# Autodesk Inventor assembly: BobbinGuide
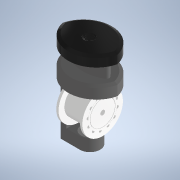
[picture p0: Inventor's stored thumbnail of the model, 180x180]
Saved by Autodesk Inventor 2022 (Build 260153000, 153)
## iProperties
Created: 2020-03-09
Part Number: BobbinGuide
Document SubType Name: Assembly
Designer: elmar
Author: elmar
## Documents named in this file (6)
- C:\repo\FourWireBraidingMachine\MetalCableBraider\Carriage.iam
- C:\repo\FourWireBraidingMachine\MetalCableBraider\CarriagePlate.ipt
- C:\repo\FourWireBraidingMachine\MetalCableBraider\SpoolHolder.ipt
- C:\repo\FourWireBraidingMachine\MetalCableBraider\Spool.ipt
- C:\repo\FourWireBraidingMachine\MetalCableBraider\Spring.ipt
- C:\repo\FourWireBraidingMachine\MetalCableBraider\SpoolSpringBushing.ipt
## Components (5 placed, 5 different names)
1. CarriagePlate:1 — Mate:6, Mate:7, Mate:8
2. SpoolHolder:1 — Insert:20, Mate:6, Mate:7, Mate:8
3. Spool:1 — Mate:1, Mate:5, Insert:20, Insert:22
4. Spring:1 — Mate:1, Mate:5
5. SpoolSpringBushing:1 — Insert:22
## Relationships (7: Mate 5, Insert 2)
- Mate:1: Spool:1 ↔ Spring:1
- Mate:5: Spool:1 ↔ Spring:1
- Insert:20: SpoolHolder:1 ↔ Spool:1
- Insert:22: Spool:1 ↔ SpoolSpringBushing:1
- Mate:6: CarriagePlate:1 ↔ SpoolHolder:1
- Mate:7: CarriagePlate:1 ↔ SpoolHolder:1
- Mate:8: CarriagePlate:1 ↔ SpoolHolder:1
